# Autodesk Inventor assembly: asse_s_tstage005
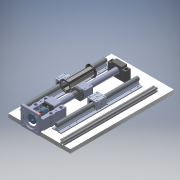
[picture p0: Inventor's stored thumbnail of the model, 180x180]
Saved by Autodesk Inventor 2019 (Build 230136000, 136)
## iProperties
Created: 2022-09-02
Part Number: asse_s_tstage005
Document SubType Name: Assembly
Designer: kananovicha
Author: kananovicha
## Documents named in this file (8)
- C:\Users\kananovicha\Documents\work\workAppState\prj_shocksL\s_tstage\drawingsGit\s_tstage\asse_s_tstage\asse_s_tstage005.iam
- C:\Users\kananovicha\Documents\work\workAppState\prj_shocksL\s_tstage\drawingsGit\s_tstage\mplate\mplate.ipt
- C:\Users\kananovicha\Documents\work\workAppState\prj_shocksL\s_tstage\drawingsGit\s_tstage\3rdParty\ballScrewAssembly\2510 L=400.iam
- C:\Users\kananovicha\Documents\work\workAppState\prj_shocksL\s_tstage\drawingsGit\s_tstage\allmainparams\allmainparams.ipt
- C:\Users\kananovicha\Documents\work\workAppState\prj_shocksL\s_tstage\drawingsGit\s_tstage\3rdParty\KF40nipple\qf40-150-n.iam
- C:\Users\kananovicha\Documents\work\workAppState\prj_shocksL\s_tstage\drawingsGit\s_tstage\3rdParty\br20-shaft-and-support-rail-resizable-1.snapshot.13\BR20\BR20-400.iam
- C:\Users\kananovicha\Documents\work\workAppState\prj_shocksL\s_tstage\drawingsGit\s_tstage\3rdParty\mod-sbr20uu-open-linear-bearing-1.snapshot.2\SBR20UU.iam
- C:\Users\kananovicha\Documents\work\workAppState\prj_shocksL\s_tstage\drawingsGit\s_tstage\tslot2020short\tslot2020short.ipt
## Components (8 placed, 6 different names)
1. mplate:1 — Flush:1, Mate:1, Mate:2, Mate:3, Mate:4, Angle:1, Angle:2, Angle:3, Flush:4, Mate:7
2. 2510 L=400:1 [sub-assembly] — Flush:1, Mate:1, Mate:2, Flush:2, Flush:3, Mate:5, Mate:6
3. qf40-150-n:1 [sub-assembly]
4. BR20-400:1 [sub-assembly] — Mate:3, Cylindrical:1, Angle:2, Flush:2, Mate:5, Mate:8
5. BR20-400:2 [sub-assembly] — Mate:4, Cylindrical:2, Flush:3, Mate:6
6. SBR20UU:1 [sub-assembly] — Cylindrical:1, Angle:1
7. SBR20UU:2 [sub-assembly] — Cylindrical:2, Angle:3
8. tslot2020short:1 — Flush:4, Mate:7, Mate:8
## Relationships (17: Mate 8, Flush 4, Angle 3, CylindricalJoint 2)
- Flush:1 (68.58 mm): mplate:1 ↔ 2510 L=400:1
- Mate:1: mplate:1 ↔ 2510 L=400:1
- Mate:2: mplate:1 ↔ 2510 L=400:1
- Mate:3: mplate:1 ↔ BR20-400:1
- Mate:4: mplate:1 ↔ BR20-400:2
- Cylindrical:1: BR20-400:1 ↔ SBR20UU:1
- Angle:1 (0 deg): mplate:1 ↔ SBR20UU:1
- Angle:2 (0 deg): mplate:1 ↔ BR20-400:1
- Cylindrical:2: BR20-400:2 ↔ SBR20UU:2
- Angle:3 (0 deg): mplate:1 ↔ SBR20UU:2
- Flush:2: 2510 L=400:1 ↔ BR20-400:1
- Flush:3: 2510 L=400:1 ↔ BR20-400:2
- Mate:5 (12.7 mm): 2510 L=400:1 ↔ BR20-400:1
- Mate:6 (12.7 mm): 2510 L=400:1 ↔ BR20-400:2
- Flush:4: mplate:1 ↔ tslot2020short:1
- Mate:7: mplate:1 ↔ tslot2020short:1
- Mate:8 (38.354 mm): BR20-400:1 ↔ tslot2020short:1
## Named parameters: asse_sfu_offset_wid = 68.58 mm, asse_sbr_railSeparation = 12.7 mm, asse_tslo_separation = 38.354 mm
